# Autodesk Inventor assembly: XY_Table_Plate
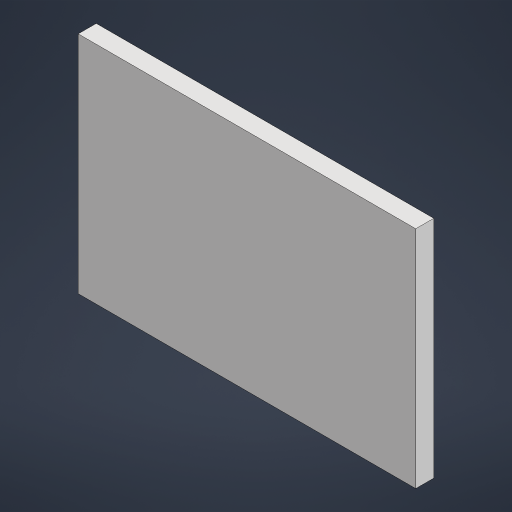
[picture p0: Inventor's stored thumbnail of the model, 512x512]
Saved by Autodesk Inventor 2024.2 (Build 282272000, 272)
## iProperties
Created: 2024-02-04
Part Number: XY_Table_Plate
Document SubType Name: Assembly
Designer: Hanaoka
Author: Hanaoka
## Documents named in this file (2)
- G:\共有ドライブ\reRo\05_個人\hanaoka\inventor\3Dprint\XY_Table_Plate.iam
- G:\共有ドライブ\reRo\05_個人\hanaoka\inventor\3Dprint\Plate.ipt
## Components (1 placed, 1 different names)
1. Plate:1 — メイト:1, メイト:2, メイト:3
## Relationships (3: Mate 3)
- メイト:1 [Mate]: Plate:1
- メイト:2 [Mate]: Plate:1
- メイト:3 [Mate]: Plate:1
